# Autodesk Inventor assembly: Base
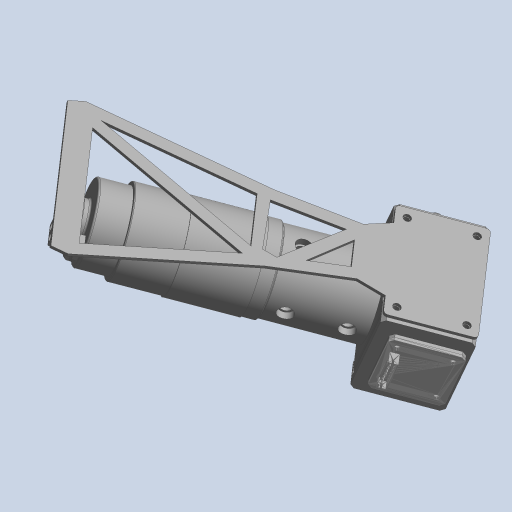
[picture p0: Inventor's stored thumbnail of the model, 512x512]
Saved by Autodesk Inventor 2023 (Build 270158000, 158)
## iProperties
Created: 2020-03-24
Part Number: Base
Document SubType Name: Assembly
Designer: valer
Mass: 715.256 g
Surface Area: 821.775 cm^2
Volume: 200.817 cm^3
Density: 3.56173 g/cm^3
Author: valer
## Documents named in this file (6)
- C:\Users\LattePanda\Desktop\str1ker\cad\ArmBase.iam
- C:\Users\LattePanda\Desktop\str1ker\cad\external\ShoulderActuator\DumaDynamics00E.ipt
- C:\Users\LattePanda\Desktop\str1ker\cad\ShoulderMotorMount.ipt
- C:\Users\LattePanda\Desktop\str1ker\cad\ShoulderEncoderSpacer.ipt
- C:\Users\LattePanda\Desktop\str1ker\cad\external\ShoulderEncoder\ArmEncoderBoard.ipt
- C:\Users\LattePanda\Desktop\str1ker\cad\ShoulderMount.ipt
## Components (6 placed, 5 different names)
1. DumaDynamics00E:1 — Mate:1, Flush:1, Mate:2, Mate:3, Mate:4
2. ShoulderMotorMount:1 — Mate:1, Mate:2, Mate:3, Flush:2, Mate:5, Mate:6, Mate:15, Flush:3
3. ShoulderMotorMount:2 — Mate:4, Mate:5, Mate:6, Mate:9, Mate:10, Mate:11
4. ShoulderEncoderSpacer:1 — Mate:9, Mate:10, Mate:11, Mate:12, Mate:13, Mate:14
5. ArmEncoderBoard:1 — Mate:12, Mate:13, Mate:14
6. ShoulderMount:1 — Flush:3
## Relationships (16: Mate 13, Flush 3)
- Mate:1: DumaDynamics00E:1 ↔ ShoulderMotorMount:1
- Flush:1: DumaDynamics00E:1
- Mate:2: DumaDynamics00E:1 ↔ ShoulderMotorMount:1
- Mate:3: DumaDynamics00E:1 ↔ ShoulderMotorMount:1
- Flush:2: ShoulderMotorMount:1
- Mate:4: DumaDynamics00E:1 ↔ ShoulderMotorMount:2
- Mate:5: ShoulderMotorMount:1 ↔ ShoulderMotorMount:2
- Mate:6: ShoulderMotorMount:1 ↔ ShoulderMotorMount:2
- Mate:9: ShoulderMotorMount:2 ↔ ShoulderEncoderSpacer:1
- Mate:10: ShoulderMotorMount:2 ↔ ShoulderEncoderSpacer:1
- Mate:11: ShoulderMotorMount:2 ↔ ShoulderEncoderSpacer:1
- Mate:12: ShoulderEncoderSpacer:1 ↔ ArmEncoderBoard:1
- Mate:13: ShoulderEncoderSpacer:1 ↔ ArmEncoderBoard:1
- Mate:14: ShoulderEncoderSpacer:1 ↔ ArmEncoderBoard:1
- Mate:15: ShoulderMotorMount:1
- Flush:3: ShoulderMotorMount:1 ↔ ShoulderMount:1
